# Autodesk Inventor assembly: sub_flap
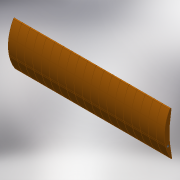
[picture p0: Inventor's stored thumbnail of the model, 180x180]
Saved by Autodesk Inventor 2018.2 (Build 222227000, 227)
## iProperties
Created: 2017-12-11
Part Number: sub_flap
Material: 一般
Document SubType Name: Assembly
Designer: kuwano
Author: kuwano
## Documents named in this file (3)
- D:\kuwano\Documents\Inventor\KITformula\AeroCAD2018\CAD\Inventor\製作用CAD\R-wing\parts\sub_flap\sub_flap.iam
- D:\kuwano\Documents\Inventor\KITformula\AeroCAD2018\CAD\Inventor\製作用CAD\R-wing\parts\sub_flap\parts\styro_50_sub.ipt
- D:\kuwano\Documents\Inventor\KITformula\AeroCAD2018\CAD\Inventor\製作用CAD\R-wing\parts\sub_flap\parts\pipe.ipt
## Components (20 placed, 2 different names)
1. styro_50_sub:1 — メイト:1, メイト:19, メイト:37, フラッシュ:2
2. styro_50_sub:2 — メイト:1, メイト:2, メイト:19, メイト:20, メイト:37, メイト:38
3. styro_50_sub:3 — メイト:2, メイト:3, メイト:20, メイト:21, メイト:38, メイト:39
4. styro_50_sub:4 — メイト:3, メイト:4, メイト:21, メイト:22, メイト:39, メイト:40
5. styro_50_sub:5 — メイト:4, メイト:5, メイト:22, メイト:23, メイト:40, メイト:41
6. styro_50_sub:6 — メイト:5, メイト:6, メイト:23, メイト:24, メイト:41, メイト:42
7. styro_50_sub:7 — メイト:6, メイト:7, メイト:24, メイト:25, メイト:42, メイト:43
8. styro_50_sub:8 — メイト:7, メイト:8, メイト:25, メイト:26, メイト:43, メイト:44
9. styro_50_sub:9 — メイト:8, メイト:9, メイト:26, メイト:27, メイト:44, メイト:45
10. styro_50_sub:10 — メイト:9, メイト:10, メイト:27, メイト:28, メイト:45, メイト:46
11. styro_50_sub:11 — メイト:10, メイト:11, メイト:28, メイト:29, メイト:46, メイト:47
12. styro_50_sub:12 — メイト:11, メイト:12, メイト:29, メイト:30, メイト:47, メイト:48
13. styro_50_sub:13 — メイト:12, メイト:13, メイト:30, メイト:31, メイト:48, メイト:49
14. styro_50_sub:14 — メイト:13, メイト:14, メイト:31, メイト:32, メイト:49, メイト:50
15. styro_50_sub:15 — メイト:14, メイト:15, メイト:32, メイト:33, メイト:50, メイト:51
16. styro_50_sub:16 — メイト:15, メイト:16, メイト:33, メイト:34, メイト:51, メイト:52
17. styro_50_sub:17 — メイト:16, メイト:17, メイト:34, メイト:35, メイト:52, メイト:53
18. styro_50_sub:18 — メイト:17, メイト:18, メイト:35, メイト:36, メイト:53, メイト:54
19. styro_50_sub:19 — メイト:18, メイト:36, メイト:54, メイト:55, フラッシュ:1
20. pipe:1 — メイト:55, フラッシュ:1, フラッシュ:2
## Relationships (57: Mate 55, Flush 2)
- メイト:1 [Mate]: styro_50_sub:1 ↔ styro_50_sub:2
- メイト:2 [Mate]: styro_50_sub:2 ↔ styro_50_sub:3
- メイト:3 [Mate]: styro_50_sub:3 ↔ styro_50_sub:4
- メイト:4 [Mate]: styro_50_sub:4 ↔ styro_50_sub:5
- メイト:5 [Mate]: styro_50_sub:5 ↔ styro_50_sub:6
- メイト:6 [Mate]: styro_50_sub:6 ↔ styro_50_sub:7
- メイト:7 [Mate]: styro_50_sub:7 ↔ styro_50_sub:8
- メイト:8 [Mate]: styro_50_sub:8 ↔ styro_50_sub:9
- メイト:9 [Mate]: styro_50_sub:9 ↔ styro_50_sub:10
- メイト:10 [Mate]: styro_50_sub:10 ↔ styro_50_sub:11
- メイト:11 [Mate]: styro_50_sub:11 ↔ styro_50_sub:12
- メイト:12 [Mate]: styro_50_sub:12 ↔ styro_50_sub:13
- メイト:13 [Mate]: styro_50_sub:13 ↔ styro_50_sub:14
- メイト:14 [Mate]: styro_50_sub:14 ↔ styro_50_sub:15
- メイト:15 [Mate]: styro_50_sub:15 ↔ styro_50_sub:16
- メイト:16 [Mate]: styro_50_sub:16 ↔ styro_50_sub:17
- メイト:17 [Mate]: styro_50_sub:17 ↔ styro_50_sub:18
- メイト:18 [Mate]: styro_50_sub:18 ↔ styro_50_sub:19
- メイト:19 [Mate]: styro_50_sub:1 ↔ styro_50_sub:2
- メイト:20 [Mate]: styro_50_sub:2 ↔ styro_50_sub:3
- メイト:21 [Mate]: styro_50_sub:3 ↔ styro_50_sub:4
- メイト:22 [Mate]: styro_50_sub:4 ↔ styro_50_sub:5
- メイト:23 [Mate]: styro_50_sub:5 ↔ styro_50_sub:6
- メイト:24 [Mate]: styro_50_sub:6 ↔ styro_50_sub:7
- メイト:25 [Mate]: styro_50_sub:7 ↔ styro_50_sub:8
- メイト:26 [Mate]: styro_50_sub:8 ↔ styro_50_sub:9
- メイト:27 [Mate]: styro_50_sub:9 ↔ styro_50_sub:10
- メイト:28 [Mate]: styro_50_sub:10 ↔ styro_50_sub:11
- メイト:29 [Mate]: styro_50_sub:11 ↔ styro_50_sub:12
- メイト:30 [Mate]: styro_50_sub:12 ↔ styro_50_sub:13
- メイト:31 [Mate]: styro_50_sub:13 ↔ styro_50_sub:14
- メイト:32 [Mate]: styro_50_sub:14 ↔ styro_50_sub:15
- メイト:33 [Mate]: styro_50_sub:15 ↔ styro_50_sub:16
- メイト:34 [Mate]: styro_50_sub:16 ↔ styro_50_sub:17
- メイト:35 [Mate]: styro_50_sub:17 ↔ styro_50_sub:18
- メイト:36 [Mate]: styro_50_sub:18 ↔ styro_50_sub:19
- メイト:37 [Mate]: styro_50_sub:1 ↔ styro_50_sub:2
- メイト:38 [Mate]: styro_50_sub:2 ↔ styro_50_sub:3
- メイト:39 [Mate]: styro_50_sub:3 ↔ styro_50_sub:4
- メイト:40 [Mate]: styro_50_sub:4 ↔ styro_50_sub:5
- メイト:41 [Mate]: styro_50_sub:5 ↔ styro_50_sub:6
- メイト:42 [Mate]: styro_50_sub:6 ↔ styro_50_sub:7
- メイト:43 [Mate]: styro_50_sub:7 ↔ styro_50_sub:8
- メイト:44 [Mate]: styro_50_sub:8 ↔ styro_50_sub:9
- メイト:45 [Mate]: styro_50_sub:9 ↔ styro_50_sub:10
- メイト:46 [Mate]: styro_50_sub:10 ↔ styro_50_sub:11
- メイト:47 [Mate]: styro_50_sub:11 ↔ styro_50_sub:12
- メイト:48 [Mate]: styro_50_sub:12 ↔ styro_50_sub:13
- メイト:49 [Mate]: styro_50_sub:13 ↔ styro_50_sub:14
- メイト:50 [Mate]: styro_50_sub:14 ↔ styro_50_sub:15
- メイト:51 [Mate]: styro_50_sub:15 ↔ styro_50_sub:16
- メイト:52 [Mate]: styro_50_sub:16 ↔ styro_50_sub:17
- メイト:53 [Mate]: styro_50_sub:17 ↔ styro_50_sub:18
- メイト:54 [Mate]: styro_50_sub:18 ↔ styro_50_sub:19
- メイト:55 [Mate]: styro_50_sub:19 ↔ pipe:1
- フラッシュ:1 [Flush]: styro_50_sub:19 ↔ pipe:1
- フラッシュ:2 [Flush]: styro_50_sub:1 ↔ pipe:1
